# Autodesk Inventor assembly: palm_plate
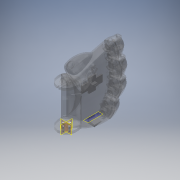
[picture p0: Inventor's stored thumbnail of the model, 180x180]
Saved by Autodesk Inventor 2019 (Build 230136000, 136)
## iProperties
Created: 2024-08-26
Part Number: palm_plate
Material: Generisch
Document SubType Name: Assembly
Designer: nic
Author: nic
## Documents named in this file (4)
- C:\Users\Nicolas Frick\Sync\OneDrive\wtm\nicol_rh8d\inventor\palm_plate.iam
- C:\Users\Nicolas Frick\Sync\OneDrive\wtm\nicol_rh8d\inventor\palm.ipt
- C:\Users\Nicolas Frick\Sync\OneDrive\wtm\nicol_rh8d\inventor\palm_plate.ipt
- C:\Users\Nicolas Frick\Sync\OneDrive\wtm\nicol_rh8d\inventor\palm_side_plate.ipt
## Components (3 placed, 3 different names)
1. palm:1 — Fluchtend:1, Passend:1
2. palm_plate:1 — Fluchtend:2, Fluchtend:3, Fluchtend:4
3. palm_side_plate:1 — Fluchtend:3, Fluchtend:5
## Relationships (6: Flush 5, Mate 1)
- Fluchtend:1 [Flush] (27.3 mm): palm:1
- Passend:1 [Mate]: palm:1
- Fluchtend:2 [Flush]: palm_plate:1
- Fluchtend:3 [Flush]: palm_plate:1 ↔ palm_side_plate:1
- Fluchtend:4 [Flush] (32 mm): palm_plate:1
- Fluchtend:5 [Flush]: palm_side_plate:1
